# Autodesk Inventor assembly: zlozenie_kompetne_WIZUAL
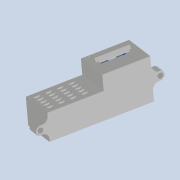
[picture p0: Inventor's stored thumbnail of the model, 180x180]
Saved by Autodesk Inventor 2021 (Build 250183000, 183)
## iProperties
Created: 2025-11-29
Part Number: zlozenie_kompetne_WIZUAL
Document SubType Name: Assembly
Designer: huber
Mass: 149.647 g
Surface Area: 1067.88 cm^2
Volume: 149.647 cm^3
Density: 1 g/cm^3
Author: huber
## Documents named in this file (3)
- C:\Users\huber\OneDrive\Pulpit\hackaton BHL\BHL 2025\zlozenie_kompetne_WIZUAL.iam
- C:\Users\huber\OneDrive\Pulpit\hackaton BHL\BHL 2025\Drawer_WIZ.iam
- C:\Users\huber\OneDrive\Pulpit\hackaton BHL\BHL 2025\obudowa_WIZ.ipt
## Components (2 placed, 2 different names)
1. Drawer_WIZ:1 [sub-assembly] — Mate:1, Flush:1, Flush:2
2. obudowa_WIZ:1 — Mate:1, Flush:1, Flush:2
## Relationships (3: Flush 2, Mate 1)
- Mate:1: Drawer_WIZ:1 ↔ obudowa_WIZ:1
- Flush:1: Drawer_WIZ:1 ↔ obudowa_WIZ:1
- Flush:2: Drawer_WIZ:1 ↔ obudowa_WIZ:1
